# Autodesk Inventor assembly: BED
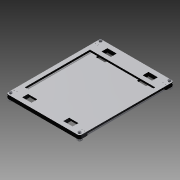
[picture p0: Inventor's stored thumbnail of the model, 180x180]
Saved by Autodesk Inventor 2013 (Build 170138000, 138)
## iProperties
Created: 2014-06-19
Part Number: BED
Document SubType Name: Assembly
Designer: employee
Author: employee
## Documents named in this file (12)
- C:\Users\employee\Desktop\CoreXZ 2\BED.iam
- C:\Users\employee\Desktop\CoreXZ 2\BED PLATE BOTTOM.ipt
- C:\Users\employee\Desktop\CoreXZ 2\M8X290 ROD.ipt
- C:\Users\employee\Desktop\CoreXZ 2\BED PLATE TOP.ipt
- C:\Users\employee\Desktop\CoreXZ 2\625vv.ipt
- C:\Users\employee\Desktop\CoreXZ 2\M5 WASHER.ipt
- C:\Users\employee\Desktop\CoreXZ 2\M5X25.ipt
- C:\Users\employee\Desktop\CoreXZ 2\M5 NUT.ipt
- C:\Users\employee\Desktop\CoreXZ 2\ZIP TIE GANTRY ROD.ipt
- C:\Users\employee\Desktop\CoreXZ 2\SILICON HEATER PAD.ipt
- C:\Users\employee\Desktop\CoreXZ 2\GLASS.ipt
- C:\Users\employee\Desktop\CoreXZ 2\BINDER CLIP.iam
## Components (30 placed, 11 different names)
1. BED PLATE BOTTOM:1 — Mate:1, Mate:2, Tangent:1, Tangent:2, Tangent:3, Tangent:4, Flush:1, Insert:1, Insert:2, Insert:3, Insert:4, Angle:1, Angle:2, Angle:3, Angle:4, Mate:15
2. M8X290 ROD:1 — Mate:1, Tangent:1, Tangent:2, Insert:17, Insert:19
3. M8X290 ROD:2 — Mate:2, Tangent:3, Tangent:4, Insert:18, Insert:20
4. BED PLATE TOP:1 — Flush:1, Insert:13, Insert:14, Insert:15, Insert:16, Mate:3, Mate:4, Flush:2, Flush:3, Flush:4, Mate:6, Mate:7, Mate:8, Mate:9, Mate:14, Mate:16, Mate:17
5. 625vv:1 — Insert:5, Insert:9
6. 625vv:2 — Insert:6, Insert:10
7. 625vv:3 — Insert:7, Insert:11
8. 625vv:4 — Insert:8, Insert:12
9. M5 WASHER:1 — Insert:1, Insert:5
10. M5 WASHER:2 — Insert:2, Insert:6
11. M5 WASHER:3 — Insert:3, Insert:7
12. M5 WASHER:4 — Insert:4, Insert:8
13. M5X25:1 — Insert:9
14. M5X25:2 — Insert:10
15. M5X25:3 — Insert:11
16. M5X25:4 — Insert:12
17. M5 NUT:1 — Insert:13
18. M5 NUT:2 — Insert:16
19. M5 NUT:3 — Insert:14
20. M5 NUT:4 — Insert:15
21. ZIP TIE GANTRY ROD:1 — Insert:17, Angle:3
22. ZIP TIE GANTRY ROD:2 — Insert:18, Angle:2
23. ZIP TIE GANTRY ROD:3 — Insert:19, Angle:4
24. ZIP TIE GANTRY ROD:4 — Insert:20, Angle:1
25. SILICON HEATER PAD:1 — Mate:3, Mate:4, Flush:2, Mate:5
26. GLASS:1 — Mate:5, Flush:3, Flush:4, Mate:10, Mate:11, Mate:12, Mate:13
27. BINDER CLIP:1 [sub-assembly] — Mate:6, Mate:12, Mate:14
28. BINDER CLIP:2 [sub-assembly] — Mate:7, Mate:13, Mate:15
29. BINDER CLIP:3 [sub-assembly] — Mate:8, Mate:10, Mate:16
30. BINDER CLIP:4 [sub-assembly] — Mate:9, Mate:11, Mate:17
## Relationships (49: Insert 20, Mate 17, Tangent 4, Flush 4, Angle 4)
- Mate:1: BED PLATE BOTTOM:1 ↔ M8X290 ROD:1
- Mate:2: BED PLATE BOTTOM:1 ↔ M8X290 ROD:2
- Tangent:1: BED PLATE BOTTOM:1 ↔ M8X290 ROD:1
- Tangent:2: BED PLATE BOTTOM:1 ↔ M8X290 ROD:1
- Tangent:3: BED PLATE BOTTOM:1 ↔ M8X290 ROD:2
- Tangent:4: BED PLATE BOTTOM:1 ↔ M8X290 ROD:2
- Flush:1: BED PLATE BOTTOM:1 ↔ BED PLATE TOP:1
- Insert:1: BED PLATE BOTTOM:1 ↔ M5 WASHER:1
- Insert:2: BED PLATE BOTTOM:1 ↔ M5 WASHER:2
- Insert:3: BED PLATE BOTTOM:1 ↔ M5 WASHER:3
- Insert:4: BED PLATE BOTTOM:1 ↔ M5 WASHER:4
- Insert:5: 625vv:1 ↔ M5 WASHER:1
- Insert:6: 625vv:2 ↔ M5 WASHER:2
- Insert:7: 625vv:3 ↔ M5 WASHER:3
- Insert:8: 625vv:4 ↔ M5 WASHER:4
- Insert:9: 625vv:1 ↔ M5X25:1
- Insert:10: 625vv:2 ↔ M5X25:2
- Insert:11: 625vv:3 ↔ M5X25:3
- Insert:12: 625vv:4 ↔ M5X25:4
- Insert:13: BED PLATE TOP:1 ↔ M5 NUT:1
- Insert:14: BED PLATE TOP:1 ↔ M5 NUT:3
- Insert:15: BED PLATE TOP:1 ↔ M5 NUT:4
- Insert:16: BED PLATE TOP:1 ↔ M5 NUT:2
- Insert:17 (3.25 mm): M8X290 ROD:1 ↔ ZIP TIE GANTRY ROD:1
- Insert:18 (3.25 mm): M8X290 ROD:2 ↔ ZIP TIE GANTRY ROD:2
- Insert:19 (3.25 mm): M8X290 ROD:1 ↔ ZIP TIE GANTRY ROD:3
- Insert:20 (3.25 mm): M8X290 ROD:2 ↔ ZIP TIE GANTRY ROD:4
- Angle:1 (0 deg): BED PLATE BOTTOM:1 ↔ ZIP TIE GANTRY ROD:4
- Angle:2 (0 deg): BED PLATE BOTTOM:1 ↔ ZIP TIE GANTRY ROD:2
- Angle:3 (0 deg): BED PLATE BOTTOM:1 ↔ ZIP TIE GANTRY ROD:1
- Angle:4 (0 deg): BED PLATE BOTTOM:1 ↔ ZIP TIE GANTRY ROD:3
- Mate:3 (0.5 mm): BED PLATE TOP:1 ↔ SILICON HEATER PAD:1
- Mate:4 (0.5 mm): BED PLATE TOP:1 ↔ SILICON HEATER PAD:1
- Flush:2: BED PLATE TOP:1 ↔ SILICON HEATER PAD:1
- Mate:5 (0.01 mm): SILICON HEATER PAD:1 ↔ GLASS:1
- Flush:3: BED PLATE TOP:1 ↔ GLASS:1
- Flush:4: BED PLATE TOP:1 ↔ GLASS:1
- Mate:6: BED PLATE TOP:1 ↔ BINDER CLIP:1
- Mate:7: BED PLATE TOP:1 ↔ BINDER CLIP:2
- Mate:8: BED PLATE TOP:1 ↔ BINDER CLIP:3
- Mate:9: BED PLATE TOP:1 ↔ BINDER CLIP:4
- Mate:10: GLASS:1 ↔ BINDER CLIP:3
- Mate:11: GLASS:1 ↔ BINDER CLIP:4
- Mate:12: GLASS:1 ↔ BINDER CLIP:1
- Mate:13: GLASS:1 ↔ BINDER CLIP:2
- Mate:14 (1.5 mm): BED PLATE TOP:1 ↔ BINDER CLIP:1
- Mate:15 (1.5 mm): BED PLATE BOTTOM:1 ↔ BINDER CLIP:2
- Mate:16 (1.5 mm): BED PLATE TOP:1 ↔ BINDER CLIP:3
- Mate:17 (1.5 mm): BED PLATE TOP:1 ↔ BINDER CLIP:4
